# Autodesk Inventor assembly: Batteriepack
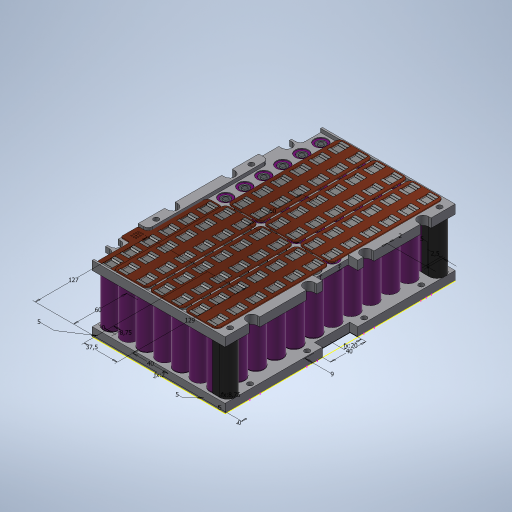
[picture p0: Inventor's stored thumbnail of the model, 512x512]
Saved by Autodesk Inventor 2024 (Build 280153000, 153)
## iProperties
Created: 2025-03-26
Part Number: Batteriepack
Document SubType Name: Assembly
Designer: David Lill
Author: David Lill
## Documents named in this file (10)
- C:\Users\Angela Ogrenda\Documents\Batterie_Konstruktion\E-16 Batterie\Batteriepack.iam
- C:\Users\Angela Ogrenda\Documents\Batterie_Konstruktion\E-16 Batterie\Platte1.ipt
- C:\Users\Angela Ogrenda\Documents\Batterie_Konstruktion\E-16 Batterie\Abstandhalter.ipt
- C:\Users\Angela Ogrenda\Documents\Batterie_Konstruktion\E-16 Batterie\Bat_contacts_v2.iam
- C:\Users\Angela Ogrenda\Documents\Batterie_Konstruktion\E-16 Batterie\18650_assembly.iam
- C:\Users\Angela Ogrenda\Documents\Batterie_Konstruktion\E-16 Batterie\Bat_contacts_v2_long.iam
- C:\Users\Angela Ogrenda\Documents\Batterie_Konstruktion\E-16 Batterie\Platine_unten.ipt
- C:\Users\Angela Ogrenda\Documents\Batterie_Konstruktion\E-16 Batterie\Bat_contacts_v2_contact.iam
- C:\Users\Angela Ogrenda\Documents\Batterie_Konstruktion\E-16 Batterie\Platine_oben.ipt
- C:\Users\Angela Ogrenda\Documents\Batterie_Konstruktion\E-16 Batterie\Platte2.ipt
## Components (23 placed, 9 different names)
1. Platte1:4 — Einfügen:11, Einfügen:12, Einfügen:13, Einfügen:16, Fluchtend:1, Passend:1, Fluchtend:4, Passend:11, Passend:13, Passend:14, Passend:17, Passend:19, Passend:21, Einfügen:18, Passend:23
2. Abstandhalter:1 — Einfügen:12
3. Abstandhalter:2 — Einfügen:11, Passend:25
4. 18650_assembly:1 [sub-assembly] — Einfügen:13, Einfügen:16, Passend:6, Passend:7, Passend:10, Einfügen:17, Passend:22, Passend:24
5. Bat_contacts_v2_long:1 [sub-assembly] — Passend:6, Tangential:1, Passend:28, Passend:29
6. Platine_unten:1 — Tangential:1
7. Bat_contacts_v2_contact:1 [sub-assembly] — Passend:10, Passend:11, Passend:12
8. Platine_oben:1 — Passend:13, Passend:14, Tangential:2
9. Platte2:1 — Einfügen:17, Passend:21, Passend:25, Passend:26, Passend:27, Passend:28, Passend:29
10. Abstandhalter:3 — Einfügen:18, Passend:22
11. Abstandhalter:4 — Passend:23, Passend:24
12. Bat_contacts_v2:1 [sub-assembly] — Fluchtend:1, Passend:1, Fluchtend:4, Passend:12
13. Bat_contacts_v2:7 [sub-assembly] — Passend:7, Passend:26, Passend:27
14. Bat_contacts_v2:2 [sub-assembly]
15. Bat_contacts_v2:8 [sub-assembly]
16. Bat_contacts_v2:3 [sub-assembly]
17. Bat_contacts_v2:9 [sub-assembly]
18. Bat_contacts_v2:4 [sub-assembly]
19. Bat_contacts_v2:10 [sub-assembly]
20. Bat_contacts_v2:5 [sub-assembly] — Tangential:2
21. Bat_contacts_v2:11 [sub-assembly]
22. Bat_contacts_v2:6 [sub-assembly]
23. Bat_contacts_v2:12 [sub-assembly]
## Component patterns: (6 elements, first: Bat_contacts_v2:1 + Bat_contacts_v2:7)
## Relationships (29: Mate 19, Insert 6, Flush 2, Tangent 2)
- Einfügen:11 [Insert]: Platte1:4 ↔ Abstandhalter:2
- Einfügen:12 [Insert]: Platte1:4 ↔ Abstandhalter:1
- Einfügen:13 [Insert]: Platte1:4 ↔ 18650_assembly:1
- Einfügen:16 [Insert]: Platte1:4 ↔ 18650_assembly:1
- Fluchtend:1 [Flush] (2 mm): Platte1:4 ↔ Bat_contacts_v2:1
- Passend:1 [Mate]: Platte1:4 ↔ Bat_contacts_v2:1
- Fluchtend:4 [Flush] (31.5 mm): Platte1:4 ↔ Bat_contacts_v2:1
- Passend:6 [Mate]: 18650_assembly:1 ↔ Bat_contacts_v2_long:1
- Passend:7 [Mate]: 18650_assembly:1 ↔ Bat_contacts_v2:7
- Tangential:1: Bat_contacts_v2_long:1 ↔ Platine_unten:1
- Passend:10 [Mate]: 18650_assembly:1 ↔ Bat_contacts_v2_contact:1
- Passend:11 [Mate]: Platte1:4 ↔ Bat_contacts_v2_contact:1
- Passend:12 [Mate] (2 mm): Bat_contacts_v2_contact:1 ↔ Bat_contacts_v2:1
- Passend:13 [Mate]: Platte1:4 ↔ Platine_oben:1
- Passend:14 [Mate]: Platte1:4 ↔ Platine_oben:1
- Tangential:2: Platine_oben:1 ↔ Bat_contacts_v2:5
- Passend:17 [Mate] (-130 mm): Platte1:4
- Passend:19 [Mate]: Platte1:4
- Einfügen:17 [Insert]: 18650_assembly:1 ↔ Platte2:1
- Passend:21 [Mate]: Platte1:4 ↔ Platte2:1
- Einfügen:18 [Insert]: Platte1:4 ↔ Abstandhalter:3
- Passend:22 [Mate]: 18650_assembly:1 ↔ Abstandhalter:3
- Passend:23 [Mate]: Platte1:4 ↔ Abstandhalter:4
- Passend:24 [Mate]: 18650_assembly:1 ↔ Abstandhalter:4
- Passend:25 [Mate]: Abstandhalter:2 ↔ Platte2:1
- Passend:26 [Mate]: Platte2:1 ↔ Bat_contacts_v2:7
- Passend:27 [Mate]: Platte2:1 ↔ Bat_contacts_v2:7
- Passend:28 [Mate]: Bat_contacts_v2_long:1 ↔ Platte2:1
- Passend:29 [Mate]: Bat_contacts_v2_long:1 ↔ Platte2:1
